# Autodesk Inventor assembly: Full_Assembly_1
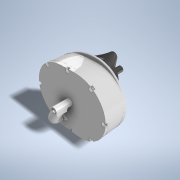
[picture p0: Inventor's stored thumbnail of the model, 180x180]
Saved by Autodesk Inventor 2021 (Build 250183000, 183)
## iProperties
Created: 2021-03-26
Part Number: Full_Assembly_1
Document SubType Name: Assembly
Designer: lucia
Author: lucia
## Documents named in this file (11)
- E:\Documents\Inventor\Fixed Rotor Wankel Engine\Assemblies\Full_Assembly_1.iam
- E:\Documents\Inventor\Fixed Rotor Wankel Engine\Parts\Rotor_Mount.ipt
- E:\Documents\Inventor\Fixed Rotor Wankel Engine\Parts\Eccentric_Shaft.ipt
- E:\Documents\Inventor\Fixed Rotor Wankel Engine\Parts\Rotor_Geared_6t_Mountable.ipt
- E:\Documents\Inventor\Fixed Rotor Wankel Engine\Parts\Side_Plate_Geared.ipt
- E:\Documents\Inventor\Fixed Rotor Wankel Engine\Parts\Housing.ipt
- E:\Documents\Inventor\Fixed Rotor Wankel Engine\Parts\Side_Plate_Intake_Exhaust.ipt
- E:\Documents\Inventor\Fixed Rotor Wankel Engine\Parts\Exhaust_Plate.ipt
- E:\Documents\Inventor\Fixed Rotor Wankel Engine\Parts\Exhaust Manifold.ipt
- E:\Documents\Inventor\Fixed Rotor Wankel Engine\Parts\Bolt Cover.ipt
- E:\Documents\Inventor\Fixed Rotor Wankel Engine\Parts\Intake Manifold.ipt
## Components (19 placed, 10 different names)
1. Rotor_Mount:1 — Mate:1, Mate:2, Mate:3, Mate:4, Flush:1, Mate:17
2. Eccentric_Shaft:1 — Mate:3, Mate:4, Mate:7, Mate:10, Rotation:1, Mate:18, Mate:38, Mate:41
3. Rotor_Geared_6t_Mountable:1 — Mate:7, Flush:1, Mate:9, Mate:17
4. Side_Plate_Geared:1 — Mate:9, Mate:10, Rotation:1, Mate:11, Mate:12, Mate:13, Mate:37, Mate:39, Mate:40
5. Housing:1 — Mate:11, Mate:12, Mate:13, Mate:14, Mate:15, Mate:16
6. Side_Plate_Intake_Exhaust:1 — Mate:14, Mate:15, Mate:16, Mate:19, Mate:29, Flush:4, Mate:30, Flush:5, Mate:31, Flush:6, Mate:32, Flush:7, Mate:33, Flush:8, Mate:34, Flush:9, Mate:35, Flush:10, Mate:36, Flush:11
7. Exhaust_Plate:1 — Mate:18, Mate:19, Mate:20, Mate:21, Mate:22, Mate:23, Mate:24, Mate:25, Mate:26, Mate:27, Mate:28
8. Exhaust Manifold:1 — Mate:20, Mate:21, Mate:22
9. Exhaust Manifold:2 — Mate:26, Mate:27, Mate:28
10. Exhaust Manifold:3 — Mate:23, Mate:24, Mate:25
11. Bolt Cover:1 — Mate:33, Flush:8
12. Bolt Cover:2 — Mate:34, Flush:9
13. Bolt Cover:3 — Mate:30, Flush:5
14. Bolt Cover:4 — Mate:32, Flush:7
15. Bolt Cover:5 — Mate:35, Flush:10
16. Bolt Cover:6 — Mate:36, Flush:11
17. Bolt Cover:7 — Mate:29, Flush:4
18. Bolt Cover:8 — Mate:31, Flush:6
19. Intake Manifold:1 — Mate:37, Mate:38, Mate:39
## Relationships (52: Mate 40, Flush 11, RelateRotation 1)
- Mate:1: Rotor_Mount:1
- Mate:2: Rotor_Mount:1
- Mate:3: Rotor_Mount:1 ↔ Eccentric_Shaft:1
- Mate:4: Rotor_Mount:1 ↔ Eccentric_Shaft:1
- Mate:7: Eccentric_Shaft:1 ↔ Rotor_Geared_6t_Mountable:1
- Flush:1: Rotor_Mount:1 ↔ Rotor_Geared_6t_Mountable:1
- Mate:9: Rotor_Geared_6t_Mountable:1 ↔ Side_Plate_Geared:1
- Mate:10: Eccentric_Shaft:1 ↔ Side_Plate_Geared:1
- Rotation:1 [RelateRotation] (0.5 ul): Eccentric_Shaft:1 ↔ Side_Plate_Geared:1
- Mate:11: Side_Plate_Geared:1 ↔ Housing:1
- Mate:12: Side_Plate_Geared:1 ↔ Housing:1
- Mate:13: Side_Plate_Geared:1 ↔ Housing:1
- Mate:14: Housing:1 ↔ Side_Plate_Intake_Exhaust:1
- Mate:15: Housing:1 ↔ Side_Plate_Intake_Exhaust:1
- Mate:16: Housing:1 ↔ Side_Plate_Intake_Exhaust:1
- Mate:17: Rotor_Mount:1 ↔ Rotor_Geared_6t_Mountable:1
- Mate:18: Eccentric_Shaft:1 ↔ Exhaust_Plate:1
- Mate:19: Side_Plate_Intake_Exhaust:1 ↔ Exhaust_Plate:1
- Mate:20: Exhaust_Plate:1 ↔ Exhaust Manifold:1
- Mate:21: Exhaust_Plate:1 ↔ Exhaust Manifold:1
- Mate:22: Exhaust_Plate:1 ↔ Exhaust Manifold:1
- Mate:23: Exhaust_Plate:1 ↔ Exhaust Manifold:3
- Mate:24: Exhaust_Plate:1 ↔ Exhaust Manifold:3
- Mate:25: Exhaust_Plate:1 ↔ Exhaust Manifold:3
- Mate:26: Exhaust_Plate:1 ↔ Exhaust Manifold:2
- Mate:27: Exhaust_Plate:1 ↔ Exhaust Manifold:2
- Mate:28: Exhaust_Plate:1 ↔ Exhaust Manifold:2
- Flush:2 (-12.7 mm)
- Flush:3 (63.5 mm)
- Mate:29: Side_Plate_Intake_Exhaust:1 ↔ Bolt Cover:7
- Flush:4: Side_Plate_Intake_Exhaust:1 ↔ Bolt Cover:7
- Mate:30: Side_Plate_Intake_Exhaust:1 ↔ Bolt Cover:3
- Flush:5: Side_Plate_Intake_Exhaust:1 ↔ Bolt Cover:3
- Mate:31: Side_Plate_Intake_Exhaust:1 ↔ Bolt Cover:8
- Flush:6: Side_Plate_Intake_Exhaust:1 ↔ Bolt Cover:8
- Mate:32: Side_Plate_Intake_Exhaust:1 ↔ Bolt Cover:4
- Flush:7: Side_Plate_Intake_Exhaust:1 ↔ Bolt Cover:4
- Mate:33: Side_Plate_Intake_Exhaust:1 ↔ Bolt Cover:1
- Flush:8: Side_Plate_Intake_Exhaust:1 ↔ Bolt Cover:1
- Mate:34: Side_Plate_Intake_Exhaust:1 ↔ Bolt Cover:2
- Flush:9: Side_Plate_Intake_Exhaust:1 ↔ Bolt Cover:2
- Mate:35: Side_Plate_Intake_Exhaust:1 ↔ Bolt Cover:5
- Flush:10: Side_Plate_Intake_Exhaust:1 ↔ Bolt Cover:5
- Mate:36: Side_Plate_Intake_Exhaust:1 ↔ Bolt Cover:6
- Flush:11: Side_Plate_Intake_Exhaust:1 ↔ Bolt Cover:6
- Mate:37: Side_Plate_Geared:1 ↔ Intake Manifold:1
- Mate:38: Eccentric_Shaft:1 ↔ Intake Manifold:1
- Mate:39: Side_Plate_Geared:1 ↔ Intake Manifold:1
- Mate:40: Side_Plate_Geared:1
- Mate:41: Eccentric_Shaft:1
- Mate:42
- Mate:43
